# Autodesk Inventor assembly: Motor-Bracket-threaded
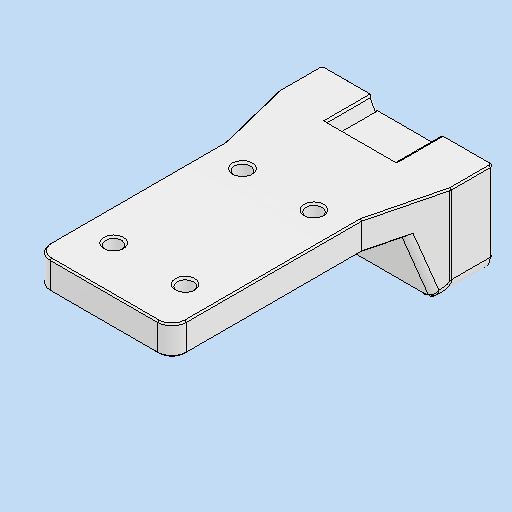
[picture p0: Inventor's stored thumbnail of the model, 512x512]
Saved by Autodesk Inventor 2025 (Build 290162000, 162)
## iProperties
Created: 2025-06-05
Part Number: Motor-Bracket-threaded
Document SubType Name: Assembly
Designer: kuzmin
Author: kuzmin
## Documents named in this file (3)
- C:\Users\queez\Dropbox\Drawings\PIHTI\LIBS\Motor-Bracket-threaded.iam
- C:\Users\queez\Dropbox\Drawings\PIHTI\LIBS\Motor-Bracket.ipt
- C:\Users\queez\Dropbox\Drawings\PIHTI\ContentCenter\Fastners\brass-insert-m3x5.ipt
## Components (5 placed, 2 different names)
1. Motor-Bracket:1
2. brass-insert-m3x5:1
3. brass-insert-m3x5:2
4. brass-insert-m3x5:3
5. brass-insert-m3x5:4
## Relationships (4: WeldJoint 4)
- [WeldJoint]: Motor-Bracket:1 ↔ brass-insert-m3x5:4
- [WeldJoint]: Motor-Bracket:1 ↔ brass-insert-m3x5:1
- [WeldJoint]: Motor-Bracket:1 ↔ brass-insert-m3x5:2
- [WeldJoint]: Motor-Bracket:1 ↔ brass-insert-m3x5:3
